# Autodesk Inventor assembly: mascon-new
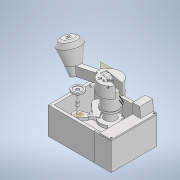
[picture p0: Inventor's stored thumbnail of the model, 180x180]
Saved by Autodesk Inventor 2021 (Build 250183000, 183)
## iProperties
Created: 2021-04-28
Part Number: mascon-new
Document SubType Name: Assembly
Designer: ben
Author: ben
## Documents named in this file (13)
- C:\Users\teh18\OneDrive\BVE Controller\r68-bve-mascon\mascon-new.iam
- C:\Users\teh18\OneDrive\BVE Controller\r68-bve-mascon\handle\handle.iam
- C:\Users\teh18\OneDrive\BVE Controller\r68-bve-mascon\shell\shell.iam
- C:\Users\teh18\OneDrive\BVE Controller\r68-bve-mascon\handle_base2.ipt
- C:\Users\teh18\OneDrive\BVE Controller\r68-bve-mascon\handle_base3.ipt
- C:\Users\teh18\OneDrive\BVE Controller\r68-bve-mascon\handle_base_rod.ipt
- C:\Users\teh18\OneDrive\BVE Controller\r68-bve-mascon\handle_base_potholder.ipt
- C:\Users\teh18\OneDrive\BVE Controller\r68-bve-mascon\handle_holder.ipt
- C:\Users\teh18\OneDrive\BVE Controller\r68-bve-mascon\Reverser.ipt
- C:\Users\teh18\OneDrive\BVE Controller\r68-bve-mascon\reverser-base.ipt
- C:\Users\teh18\OneDrive\BVE Controller\r68-bve-mascon\NotchClickerAsm.iam
- C:\Users\teh18\OneDrive\BVE Controller\r68-bve-mascon\ReverserNotch\ReverserClickAsm.iam
- C:\Users\teh18\OneDrive\BVE Controller\r68-bve-mascon\handle-base\handle_base.iam
## Components (12 placed, 12 different names)
1. shell:1 [sub-assembly] — Flush:4, Mate:12, Mate:13, Mate:14, Mate:15
2. handle_base2:1 — Flush:1, Mate:11
3. handle_base3:1 — Flush:1, Flush:2
4. handle_base_rod:1 — Mate:11
5. handle_base_potholder:1 — Flush:2
6. handle_holder:1 — Mate:16, Mate:17, Mate:18
7. Reverser:1 — Flush:4, Flush:5
8. reverser-base:1 — Flush:5, Flush:6, Flush:7
9. NotchClickerAsm:1 [sub-assembly] — Mate:12
10. ReverserClickAsm:1 [sub-assembly] — Mate:13
11. handle:1 [sub-assembly] — Mate:18
12. handle_base:1 [sub-assembly] — Mate:14, Mate:15, Mate:16, Mate:17
## Relationships (14: Mate 8, Flush 6)
- Flush:1: handle_base2:1 ↔ handle_base3:1
- Flush:2: handle_base3:1 ↔ handle_base_potholder:1
- Flush:4: shell:1 ↔ Reverser:1
- Flush:5: Reverser:1 ↔ reverser-base:1
- Mate:11: handle_base2:1 ↔ handle_base_rod:1
- Mate:12: shell:1 ↔ NotchClickerAsm:1
- Flush:6 (-36.375 mm): reverser-base:1
- Flush:7: reverser-base:1
- Mate:13: shell:1 ↔ ReverserClickAsm:1
- Mate:14: shell:1 ↔ handle_base:1
- Mate:15: shell:1 ↔ handle_base:1
- Mate:16: handle_holder:1 ↔ handle_base:1
- Mate:17: handle_holder:1 ↔ handle_base:1
- Mate:18: handle_holder:1 ↔ handle:1
